# Autodesk Inventor assembly: Ensemble1
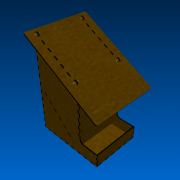
[picture p0: Inventor's stored thumbnail of the model, 180x180]
Saved by Autodesk Inventor 2013 SP2 (Build 170200200, 200)
## iProperties
Created: 2015-09-15
Part Number: Ensemble1
Document SubType Name: Assembly
Designer: jeanfrancois
Author: jeanfrancois
## Documents named in this file (9)
- E:\Inventor\Mangeoir\Ensemble1.iam
- E:\Inventor\Mangeoir\fond.ipt
- E:\Inventor\Mangeoir\devant.ipt
- E:\Inventor\Mangeoir\cote.ipt
- E:\Inventor\Mangeoir\incline.ipt
- E:\Inventor\Mangeoir\toit.ipt
- E:\Inventor\Mangeoir\Avant.ipt
- E:\Inventor\Mangeoir\Arriere.ipt
- E:\Inventor\Mangeoir\goupille.ipt
## Components (12 placed, 8 different names)
1. fond:1 — Affleurement:1, Affleurement:2, Placage:1, Placage:2, Placage:3, Affleurement:13
2. devant:1 — Affleurement:1, Affleurement:2, Placage:1, Affleurement:3, Affleurement:4, Affleurement:5, Affleurement:6
3. cote:1 — Placage:3, Affleurement:5, Affleurement:6, Placage:5, Placage:6, Placage:8, Placage:9, Placage:14, Affleurement:16, Placage:15, Affleurement:17
4. cote:2 — Placage:2, Affleurement:3, Affleurement:4, Placage:4, Placage:7, Placage:10, Affleurement:10, Placage:11, Affleurement:11, Affleurement:12, Placage:12, Affleurement:14, Placage:13, Affleurement:15
5. incline:1 — Placage:4, Placage:5, Placage:6
6. toit:1 — Placage:7, Placage:8, Placage:9
7. Avant:1 — Placage:10, Affleurement:10, Placage:11
8. Arriere:1 — Affleurement:11, Affleurement:12, Affleurement:13
9. goupille:1 — Placage:12, Affleurement:14
10. goupille:2 — Placage:14, Affleurement:16
11. goupille:3 — Placage:15, Affleurement:17
12. goupille:4 — Placage:13, Affleurement:15
## Relationships (29: Mate 15, Flush 14)
- Affleurement:1 [Flush]: fond:1 ↔ devant:1
- Affleurement:2 [Flush]: fond:1 ↔ devant:1
- Placage:1 [Mate]: fond:1 ↔ devant:1
- Placage:2 [Mate]: fond:1 ↔ cote:2
- Affleurement:3 [Flush]: devant:1 ↔ cote:2
- Affleurement:4 [Flush]: devant:1 ↔ cote:2
- Placage:3 [Mate]: fond:1 ↔ cote:1
- Affleurement:5 [Flush]: devant:1 ↔ cote:1
- Affleurement:6 [Flush]: devant:1 ↔ cote:1
- Placage:4 [Mate]: cote:2 ↔ incline:1
- Placage:5 [Mate]: cote:1 ↔ incline:1
- Placage:6 [Mate]: cote:1 ↔ incline:1
- Placage:7 [Mate]: cote:2 ↔ toit:1
- Placage:8 [Mate]: cote:1 ↔ toit:1
- Placage:9 [Mate]: cote:1 ↔ toit:1
- Placage:10 [Mate]: cote:2 ↔ Avant:1
- Affleurement:10 [Flush]: cote:2 ↔ Avant:1
- Placage:11 [Mate]: cote:2 ↔ Avant:1
- Affleurement:11 [Flush]: cote:2 ↔ Arriere:1
- Affleurement:12 [Flush]: cote:2 ↔ Arriere:1
- Affleurement:13 [Flush]: fond:1 ↔ Arriere:1
- Placage:12 [Mate]: cote:2 ↔ goupille:1
- Affleurement:14 [Flush] (-6 mm): cote:2 ↔ goupille:1
- Placage:13 [Mate]: cote:2 ↔ goupille:4
- Affleurement:15 [Flush] (6 mm): cote:2 ↔ goupille:4
- Placage:14 [Mate]: cote:1 ↔ goupille:2
- Affleurement:16 [Flush] (6 mm): cote:1 ↔ goupille:2
- Placage:15 [Mate]: cote:1 ↔ goupille:3
- Affleurement:17 [Flush] (6 mm): cote:1 ↔ goupille:3
